# Autodesk Inventor assembly: sideskirt_mount_lower
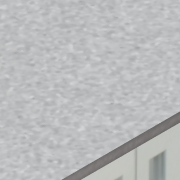
[picture p0: Inventor's stored thumbnail of the model, 180x180]
Saved by Autodesk Inventor 2016 SP2 (Build 200236200, 236)
## iProperties
Created: 2017-08-29
Part Number: sideskirt_mount_lower
Document SubType Name: Assembly
Designer: Admin
Mass: 2368.62 g
Surface Area: 6005.66 cm^2
Volume: 3154.86 cm^3
Density: 0.750784 g/cm^3
Author: Admin
## Documents named in this file (8)
- E:\DATA\Inventor\AtongJali_v2\sideskirt_mount_lower.iam
- E:\DATA\Inventor\AtongJali_v2\stepper_mount_R_1.ipt
- E:\DATA\Inventor\AtongJali_v2\base_plate_1.ipt
- E:\DATA\Inventor\AtongJali_v2\step_mount_center_1.ipt
- E:\DATA\Inventor\AtongJali_v2\step_mount_top_1.ipt
- E:\DATA\Inventor\AtongJali_v2\step_mount_front_1.ipt
- E:\DATA\Inventor\AtongJali_v2\stepper_mount_L_1.ipt
- E:\DATA\Inventor\AtongJali_v2\Linear_pipe.ipt
## Components (10 placed, 7 different names)
1. stepper_mount_R_1:1 — Rigid:1, Rigid:4
2. base_plate_1:1
3. step_mount_center_1:1
4. step_mount_top_1:1
5. step_mount_front_1:1
6. stepper_mount_L_1:1 — Rigid:2, Rigid:3
7. Linear_pipe:1 — Rigid:3
8. Linear_pipe:2 — Rigid:4
9. Linear_pipe:3 — Rigid:1
10. Linear_pipe:4 — Rigid:2
## Relationships (4: WeldJoint 4)
- Rigid:1 [WeldJoint]: stepper_mount_R_1:1 ↔ Linear_pipe:3
- Rigid:2 [WeldJoint]: stepper_mount_L_1:1 ↔ Linear_pipe:4
- Rigid:3 [WeldJoint]: stepper_mount_L_1:1 ↔ Linear_pipe:1
- Rigid:4 [WeldJoint]: stepper_mount_R_1:1 ↔ Linear_pipe:2
